# Autodesk Inventor assembly: Robot_Triciclo_(assembled_front_wheels)
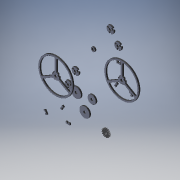
[picture p0: Inventor's stored thumbnail of the model, 180x180]
Saved by Autodesk Inventor 2019 (Build 230136000, 136)
## iProperties
Created: 2019-11-11
Part Number: Robot_Triciclo_(assembled_front_wheels)
Document SubType Name: Assembly
Designer: Domenico
Author: Domenico
Revision Number: ANY
## Documents named in this file (8)
- C:\Users\Domenico\Documents\Inventor\Mecanismos2\Robot_Triciclo_(assembled_front_wheels).iam
- C:\Users\Domenico\Documents\Inventor\Mecanismos2\Robot_Triciclo_(gear2)_Gear Blank.ipt
- C:\Users\Domenico\Documents\Inventor\Mecanismos2\Robot_Triciclo_(wheel1).ipt
- C:\Users\Domenico\Documents\Inventor\Mecanismos2\Robot_Triciclo_(wheel2).ipt
- C:\Users\Domenico\Documents\Inventor\Mecanismos2\Robot_Triciclo_(bike07).ipt
- C:\Users\Domenico\Documents\Inventor\Mecanismos2\Robot_Triciclo_(bike13).ipt
- C:\Users\Domenico\Documents\Inventor\Mecanismos2\Robot_Triciclo_(bike15).ipt
- C:\Users\Domenico\Documents\Inventor\Mecanismos2\Robot_Triciclo_(bike16).ipt
## Components (17 placed, 17 different names)
1. Robot_Triciclo_(gear2)_Gear Blank_27
2. Robot_Triciclo_(wheel1)_29 — Mate:4, Mate:5, Mate:6
3. Robot_Triciclo_(wheel1)_30 — Mate:1, Mate:2, Mate:3
4. Robot_Triciclo_(wheel2)_31
5. Robot_Triciclo_(wheel2)_32
6. Robot_Triciclo_(wheel2)_33
7. Robot_Triciclo_(wheel2)_34
8. Robot_Triciclo_(bike07)_35 — Mate:5
9. Robot_Triciclo_(bike07)_36 — Mate:4
10. Robot_Triciclo_(bike07)_37 — Mate:6
11. Robot_Triciclo_(bike07)_38 — Mate:1
12. Robot_Triciclo_(bike07)_39 — Mate:3
13. Robot_Triciclo_(bike07)_40 — Mate:2
14. Robot_Triciclo_(bike13)_41
15. Robot_Triciclo_(bike15)_42
16. Robot_Triciclo_(bike16)_43
17. Robot_Triciclo_(bike16)_44
## Relationships (6: Mate 6)
- Mate:1: Robot_Triciclo_(wheel1)_30 ↔ Robot_Triciclo_(bike07)_38
- Mate:2: Robot_Triciclo_(wheel1)_30 ↔ Robot_Triciclo_(bike07)_40
- Mate:3: Robot_Triciclo_(wheel1)_30 ↔ Robot_Triciclo_(bike07)_39
- Mate:4: Robot_Triciclo_(wheel1)_29 ↔ Robot_Triciclo_(bike07)_36
- Mate:5: Robot_Triciclo_(wheel1)_29 ↔ Robot_Triciclo_(bike07)_35
- Mate:6: Robot_Triciclo_(wheel1)_29 ↔ Robot_Triciclo_(bike07)_37
